# Autodesk Inventor assembly: Assembly1
(part 8 of 8)
